# Autodesk Inventor assembly: RFID_holder_2piece
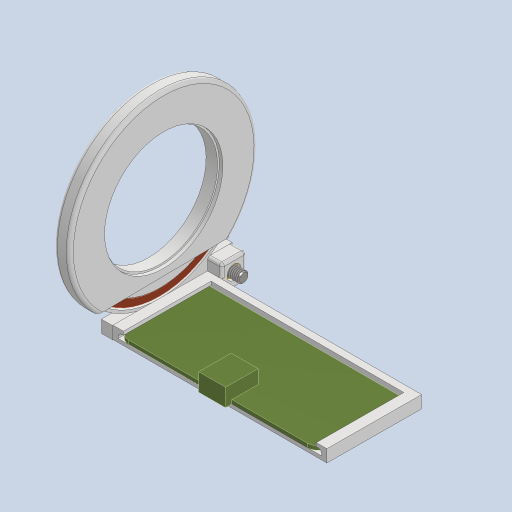
[picture p0: Inventor's stored thumbnail of the model, 512x512]
Saved by Autodesk Inventor 2024.4 (Build 284460000, 460)
## iProperties
Created: 2026-04-24
Part Number: RFID_holder_2piece
Document SubType Name: Assembly
Designer: tooles01
Author: tooles01
## Documents named in this file (8)
- C:\Users\tooles01\NYU Langone Health Dropbox\Shannon Toole\Shannon_Dropbox\Mar lab\RFID\CAD\RFID_holder\RFID_holder_2piece.iam
- C:\Users\tooles01\NYU Langone Health Dropbox\Shannon Toole\Shannon_Dropbox\Mar lab\RFID\CAD\RFID_holder\RFID_holder_coil_01.ipt
- C:\Users\tooles01\NYU Langone Health Dropbox\Shannon Toole\Shannon_Dropbox\Mar lab\RFID\CAD\lib\PCB.ipt
- C:\Users\tooles01\NYU Langone Health Dropbox\Shannon Toole\Shannon_Dropbox\Mar lab\RFID\CAD\lib\RFID_coil.ipt
- C:\Users\tooles01\NYU Langone Health Dropbox\Shannon Toole\Shannon_Dropbox\Mar lab\RFID\CAD\lib\M3 heat-set insert.ipt
- C:\Users\tooles01\Documents\Inventor\Content Center Files\R2024\en-US\AS 1420\AS 1420 - 1973 - M3 x 10.ipt
- C:\Users\tooles01\NYU Langone Health Dropbox\Shannon Toole\Shannon_Dropbox\Mar lab\RFID\CAD\RFID_holder\RFID_cover_02.ipt
- C:\Users\tooles01\NYU Langone Health Dropbox\Shannon Toole\Shannon_Dropbox\Mar lab\RFID\CAD\RFID_holder\RFID_holder_PCB_01.ipt
## Components (7 placed, 7 different names)
1. RFID_holder_coil_01:1 — coil to holder:1, screw to coil, PCB piece flush to coil piece, RFID cover to holder:face, RFID cover to holder:outside
2. RFID_holder_PCB_01:1 — PCB to holder base:1, PCB to holder back:1, PCB to holder side:1, heat-set insert to PCB piece, PCB piece flush to coil piece
3. PCB:1 — PCB to holder base:1, PCB to holder back:1, PCB to holder side:1
4. RFID_coil:1 — coil to holder:1
5. M3 heat-set insert:1 — heat-set insert to PCB piece, screw to heat-set
6. AS 1420 - Metric M3 x 10:1 — screw to coil, screw to heat-set
7. RFID_cover_02:1 — RFID cover to holder:face, RFID cover to holder:outside
## Relationships (10: Mate 7, Insert 3)
- coil to holder:1 [Insert]: RFID_holder_coil_01:1 ↔ RFID_coil:1
- PCB to holder base:1 [Mate]: RFID_holder_PCB_01:1 ↔ PCB:1
- PCB to holder back:1 [Mate]: RFID_holder_PCB_01:1 ↔ PCB:1
- PCB to holder side:1 [Mate] (1 mm): RFID_holder_PCB_01:1 ↔ PCB:1
- heat-set insert to PCB piece [Insert]: RFID_holder_PCB_01:1 ↔ M3 heat-set insert:1
- screw to coil [Insert]: RFID_holder_coil_01:1 ↔ AS 1420 - Metric M3 x 10:1
- screw to heat-set [Mate]: M3 heat-set insert:1 ↔ AS 1420 - Metric M3 x 10:1
- PCB piece flush to coil piece [Mate]: RFID_holder_coil_01:1 ↔ RFID_holder_PCB_01:1
- RFID cover to holder:face [Mate]: RFID_holder_coil_01:1 ↔ RFID_cover_02:1
- RFID cover to holder:outside [Mate]: RFID_holder_coil_01:1 ↔ RFID_cover_02:1
